# Autodesk Inventor assembly: lider
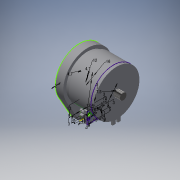
[picture p0: Inventor's stored thumbnail of the model, 180x180]
Saved by Autodesk Inventor 2018 (Build 220112000, 112)
## iProperties
Created: 2019-10-09
Part Number: lider
Material: 一般
Document SubType Name: Assembly
Designer: Eiji Nishizawa
Author: Eiji Nishizawa
## Documents named in this file (13)
- C:\Users\Eiji Nishizawa\OneDrive\CAD\二輪足回り\lider\lider.iam
- C:\Users\Eiji Nishizawa\OneDrive\CAD\二輪足回り\lider\BasePart.ipt
- C:\Users\Eiji Nishizawa\OneDrive\CAD\二輪足回り\lider\microservo.ipt
- C:\Users\Eiji Nishizawa\OneDrive\CAD\二輪足回り\lider\maingear.ipt
- C:\Users\Eiji Nishizawa\OneDrive\CAD\二輪足回り\lider\slipring.ipt
- C:\Users\Eiji Nishizawa\OneDrive\CAD\二輪足回り\lider\subgear.ipt
- C:\Users\Eiji Nishizawa\OneDrive\CAD\二輪足回り\lider\turn1part.ipt
- C:\Users\Eiji Nishizawa\OneDrive\CAD\二輪足回り\lider\sensor.ipt
- C:\Users\Eiji Nishizawa\OneDrive\CAD\二輪足回り\lider\turn2Part.ipt
- C:\Users\Eiji Nishizawa\OneDrive\CAD\二輪足回り\lider\encoder.ipt
- C:\Users\Eiji Nishizawa\OneDrive\CAD\二輪足回り\lider\encoderaxis.ipt
- C:\Users\Eiji Nishizawa\OneDrive\CAD\二輪足回り\lider\toppart.ipt
- C:\Users\Eiji Nishizawa\OneDrive\CAD\二輪足回り\lider\base_topPart.ipt
## Components (12 placed, 12 different names)
1. BasePart:1 — 挿入:1, 挿入:5, 挿入:7, フラッシュ:1, フラッシュ:2, フラッシュ:3, フラッシュ:4, メイト:1, 挿入:23, 挿入:24, 挿入:25, 挿入:26
2. microservo:1 — 挿入:1, 挿入:4, 挿入:5, フラッシュ:1, フラッシュ:2, フラッシュ:3, フラッシュ:4, メイト:1
3. maingear:1 — 挿入:6, 挿入:8
4. slipring:1 — 挿入:6, 挿入:7
5. subgear:1 — 挿入:4
6. turn1part:1 — 挿入:8, 挿入:9, 挿入:10, メイト:2, 挿入:21
7. sensor:1 — 挿入:9, 挿入:10
8. turn2Part:1 — 挿入:11, 挿入:12, 挿入:13, 挿入:14, 挿入:15, 挿入:16, 挿入:17, 挿入:18, 挿入:19, 挿入:20, メイト:2, 挿入:21, 挿入:22
9. encoder:1 — 挿入:12, 挿入:13, 挿入:15, 挿入:16, 挿入:17, 挿入:18, 挿入:19, 挿入:20
10. encoderaxis:1 — 挿入:11, 挿入:14
11. toppart:1 — 挿入:22
12. base_topPart:1 — 挿入:23, 挿入:24, 挿入:25, 挿入:26
## Relationships (30: Insert 24, Flush 4, Mate 2)
- 挿入:1 [Insert]: BasePart:1 ↔ microservo:1
- 挿入:4 [Insert]: microservo:1 ↔ subgear:1
- 挿入:5 [Insert]: BasePart:1 ↔ microservo:1
- 挿入:6 [Insert]: maingear:1 ↔ slipring:1
- 挿入:7 [Insert]: BasePart:1 ↔ slipring:1
- 挿入:8 [Insert]: maingear:1 ↔ turn1part:1
- フラッシュ:1 [Flush]: BasePart:1 ↔ microservo:1
- フラッシュ:2 [Flush]: BasePart:1 ↔ microservo:1
- フラッシュ:3 [Flush]: BasePart:1 ↔ microservo:1
- 挿入:9 [Insert]: turn1part:1 ↔ sensor:1
- 挿入:10 [Insert]: turn1part:1 ↔ sensor:1
- フラッシュ:4 [Flush]: BasePart:1 ↔ microservo:1
- メイト:1 [Mate]: BasePart:1 ↔ microservo:1
- 挿入:11 [Insert]: turn2Part:1 ↔ encoderaxis:1
- 挿入:12 [Insert]: turn2Part:1 ↔ encoder:1
- 挿入:13 [Insert]: turn2Part:1 ↔ encoder:1
- 挿入:14 [Insert]: turn2Part:1 ↔ encoderaxis:1
- 挿入:15 [Insert]: turn2Part:1 ↔ encoder:1
- 挿入:16 [Insert]: turn2Part:1 ↔ encoder:1
- 挿入:17 [Insert]: turn2Part:1 ↔ encoder:1
- 挿入:18 [Insert]: turn2Part:1 ↔ encoder:1
- 挿入:19 [Insert]: turn2Part:1 ↔ encoder:1
- 挿入:20 [Insert]: turn2Part:1 ↔ encoder:1
- メイト:2 [Mate]: turn1part:1 ↔ turn2Part:1
- 挿入:21 [Insert]: turn1part:1 ↔ turn2Part:1
- 挿入:22 [Insert]: turn2Part:1 ↔ toppart:1
- 挿入:23 [Insert]: BasePart:1 ↔ base_topPart:1
- 挿入:24 [Insert]: BasePart:1 ↔ base_topPart:1
- 挿入:25 [Insert]: BasePart:1 ↔ base_topPart:1
- 挿入:26 [Insert]: BasePart:1 ↔ base_topPart:1
